# Autodesk Inventor assembly: Assembly3
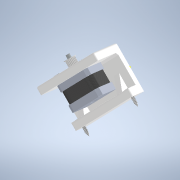
[picture p0: Inventor's stored thumbnail of the model, 180x180]
Saved by Autodesk Inventor 2021 (Build 250183000, 183)
## iProperties
Created: 2021-07-13
Part Number: Assembly3
Document SubType Name: Assembly
Designer: Michael Swaminathan
Author: Michael Swaminathan
## Documents named in this file (5)
- F:\Pattern Drawing Bot\Xy plotter Drawing Machine\Motor With Support Assembly.iam
- F:\Pattern Drawing Bot\Xy plotter Drawing Machine\X-axis.ipt
- F:\Pattern Drawing Bot\Xy plotter Drawing Machine\Servo Motor With Casing.ipt
- F:\Pattern Drawing Bot\Xy plotter Drawing Machine\Rollers.ipt
- F:\Pattern Drawing Bot\Xy plotter Drawing Machine\Screw.ipt
## Components (9 placed, 4 different names)
1. X-axis:1 — Rotational:1, Rotational:2, Rotational:3, Rotational:4, Rotational:5, Rotational:6, Rotational:7, Rotational:8
2. Servo Motor With Casing:1 — Rotational:1
3. Rollers:1 — Rotational:2
4. Screw:1 — Rotational:3
5. Screw:2 — Rotational:6
6. Screw:3 — Rotational:8
7. Screw:4 — Rotational:7
8. Screw:5 — Rotational:5
9. Screw:6 — Rotational:4
## Relationships (8: RevoluteJoint 8)
- Rotational:1 [RevoluteJoint] (-2 mm): X-axis:1 ↔ Servo Motor With Casing:1
- Rotational:2 [RevoluteJoint] (-1 mm): X-axis:1 ↔ Rollers:1
- Rotational:3 [RevoluteJoint]: X-axis:1 ↔ Screw:1
- Rotational:4 [RevoluteJoint]: X-axis:1 ↔ Screw:6
- Rotational:5 [RevoluteJoint]: X-axis:1 ↔ Screw:5
- Rotational:6 [RevoluteJoint]: X-axis:1 ↔ Screw:2
- Rotational:7 [RevoluteJoint]: X-axis:1 ↔ Screw:4
- Rotational:8 [RevoluteJoint]: X-axis:1 ↔ Screw:3
